# Autodesk Inventor assembly: Headplate_Holder_FR
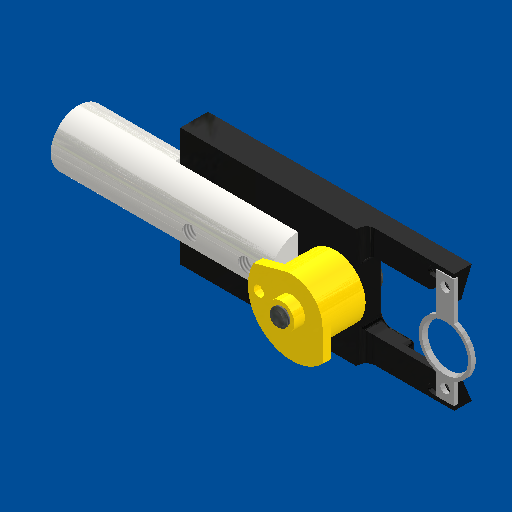
[picture p0: Inventor's stored thumbnail of the model, 512x512]
Saved by Autodesk Inventor 2025 (Build 290162000, 162)
## iProperties
Created: 2024-04-30
Part Number: Headplate_Holder_FR
Document SubType Name: Assembly
Designer: AdminForWorker
Title: Headplate_Holder_FR v11
Author: AdminForWorker
## Documents named in this file (7)
- C:\Users\faricci\Inventor\Headframe_federico\Headplate_Holder_FR v11\Headplate_Holder_FR.iam
- C:\Users\faricci\Inventor\Headframe_federico\Headplate_Holder_FR v11\Cerebellum_Headplate_new v4.ipt
- C:\Users\faricci\Inventor\Headframe_federico\Headplate_Holder_FR v11\2pConeSwivel v1.ipt
- C:\Users\faricci\Inventor\Headframe_federico\Headplate_Holder_FR v11\Part6.ipt
- C:\Users\faricci\Inventor\Headframe_federico\Headplate_Holder_FR v11\TR75T_M-Step.ipt
- C:\Users\faricci\OneDrive - Fondazione Istituto Italiano Tecnologia\Documents\Inventor\Content Center Files\R2025\en-US\ISO 7046-1 Z(1)\ISO 7046-1 - M4 x 8_ - 4.8 - Z - ISO.ipt
- C:\Users\faricci\OneDrive - Fondazione Istituto Italiano Tecnologia\Documents\Inventor\Content Center Files\R2025\en-US\ISO 7046-1 Z(1)\ISO 7046-1 - M4 x 20_ - 4.8 - Z - ISO.ipt
## Components (7 placed, 6 different names)
1. Cerebellum_Headplate_new v4:1
2. 2pConeSwivel v1:1 — Rigid:1
3. Part6 — Rigid:1, Rigid:2, Mate:1, Mate:2, Mate:3
4. TR75T_M-Step:1 — Rigid:2
5. ISO 7046-1 Z M4 x 8 - 4.8 - Z:1 — Mate:1
6. ISO 7046-1 Z M4 x 8 - 4.8 - Z:2 — Mate:2
7. ISO 7046-1 Z M4 x 20 - 4.8 - Z:1 — Mate:3
## Relationships (5: Mate 3, WeldJoint 2)
- Rigid:1 [WeldJoint]: 2pConeSwivel v1:1 ↔ Part6
- Rigid:2 [WeldJoint]: Part6 ↔ TR75T_M-Step:1
- Mate:1: Part6 ↔ ISO 7046-1 Z M4 x 8 - 4.8 - Z:1
- Mate:2: Part6 ↔ ISO 7046-1 Z M4 x 8 - 4.8 - Z:2
- Mate:3: Part6 ↔ ISO 7046-1 Z M4 x 20 - 4.8 - Z:1
